# Autodesk Inventor assembly: Pully 23mmx12mm
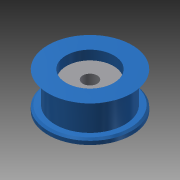
[picture p0: Inventor's stored thumbnail of the model, 180x180]
Saved by Autodesk Inventor 2013 SP2 (Build 170200200, 200)
## iProperties
Created: 2017-02-16
Part Number: Pully 23mmx12mm
Document SubType Name: Assembly
Designer: Herman de Vries
Mass: 2.51105 g
Surface Area: 23.6437 cm^2
Volume: 2.51105 cm^3
Density: 1 g/cm^3
Author: Herman de Vries
## Documents named in this file (3)
- C:\Users\hdv\Dropbox\Projects\Inventor\PaintBot_3\Pully 23mmx12mm.iam
- C:\Users\hdv\Dropbox\Projects\Inventor\PaintBot_3\bearing 4mmx13mmx5mm.ipt
- C:\Users\hdv\Dropbox\Projects\Inventor\PaintBot_3\pully13mmx23mmx12mm.ipt
## Components (2 placed, 2 different names)
1. bearing 4mmx13mmx5mm:1 — Insert:1
2. pully13mmx23mmx12mm:1 — Insert:1
## Relationships (1: Insert 1)
- Insert:1: bearing 4mmx13mmx5mm:1 ↔ pully13mmx23mmx12mm:1
